# Autodesk Inventor assembly: Wrist_B
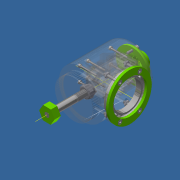
[picture p0: Inventor's stored thumbnail of the model, 180x180]
Saved by Autodesk Inventor 2016 (Build 200138000, 138)
## iProperties
Created: 2015-09-09
Part Number: Wrist_B
Material: Generisch
Document SubType Name: Assembly
Designer: 4ndreas
Mass: 237.443 g
Surface Area: 675.812 cm^2
Volume: 163.226 cm^3
Density: 1.45469 g/cm^3
Author: 4ndreas
## Documents named in this file (14)
- C:\Users\4ndreas\Documents\Inventor\RobotARM v2\v4\_assemblys\WristRot.iam
- C:\Users\4ndreas\Documents\Inventor\Content Center Files\R2014\de-DE\DIN BEARING(1)\DIN 625 SKF - SKF 61807.ipt
- C:\Users\4ndreas\Documents\Inventor\RobotARM v2\v4\_printed parts\60zGelenk.ipt
- C:\Users\4ndreas\Documents\Inventor\RobotARM v2\v4\_motors\[HerkuleX] DRS-010X.iam
- C:\Users\4ndreas\Documents\Inventor\Content Center Files\R2014\de-DE\DIN 912\DIN 912 - M2 x 0,4 x 20 x 19.ipt
- C:\Users\4ndreas\Documents\Inventor\Content Center Files\R2014\de-DE\DIN 912\DIN 912 - M3 x 0,5 x 10 x 8,75.ipt
- C:\Users\4ndreas\Documents\Inventor\Content Center Files\R2014\de-DE\DIN 985\DIN 985 - M8.ipt
- C:\Users\4ndreas\Documents\Inventor\RobotARM v2\v4\_encoder\EncoderMagnet.ipt
- C:\Users\4ndreas\Documents\Inventor\RobotARM v2\v4\_printed parts\Wrist_Cover_2.ipt
- C:\Users\4ndreas\Documents\Inventor\RobotARM v2\v4\_printed parts\magHexMount.ipt
- C:\Users\4ndreas\Documents\Inventor\Content Center Files\R2014\de-DE\DIN 931-1\DIN 931-1 - M8 x 50.ipt
- C:\Users\4ndreas\Documents\Inventor\Content Center Files\R2014\de-DE\DIN 934\DIN 934 - M3 x 0,5.ipt
- C:\Users\4ndreas\Documents\Inventor\RobotARM v2\v4\_printed parts\WristBearingHolder.ipt
- C:\Users\4ndreas\Documents\Inventor\Content Center Files\R2014\de-DE\DIN 7991(2)\DIN 7991 - M3x20.ipt
## Components (25 placed, 13 different names)
1. 60zGelenk:1 — Passend:1, Passend:2, Passend:3, Fluchtend:1, Fluchtend:2, Fluchtend:3, Passend:8, Passend:9, Passend:10, Passend:11, Passend:12, Passend:13, Passend:14, Passend:15, Passend:16, Passend:17, Passend:18, Passend:19, Fluchtend:4, Passend:29, Passend:30, Passend:33, Passend:34, Passend:36, Winkel:2, Passend:38, Passend:39, Passend:45, Passend:46, Passend:48, Passend:49, Passend:50, Passend:51, Passend:52, Passend:53, Passend:54, Passend:55, Passend:56, Fluchtend:8
2. DIN 625 SKF SKF 61807:1 — Passend:1, Passend:2, Passend:4, Passend:29, Passend:30, Passend:62
3. [HerkuleX] DRS-010X:1 [sub-assembly] — Passend:5, Fluchtend:1, Winkel:1
4. DIN 912 - ersetzt durch DIN EN ISO 4762 M2 x 20:1 — Passend:8, Passend:19
5. DIN 912 - ersetzt durch DIN EN ISO 4762 M2 x 20:2 — Passend:9, Passend:18
6. DIN 912 - ersetzt durch DIN EN ISO 4762 M2 x 20:3 — Passend:10, Passend:17
7. DIN 912 - ersetzt durch DIN EN ISO 4762 M2 x 20:4 — Passend:11, Passend:14
8. DIN 912 - ersetzt durch DIN EN ISO 4762 M2 x 20:5 — Passend:13, Passend:16
9. DIN 912 - ersetzt durch DIN EN ISO 4762 M2 x 20:6 — Passend:12, Passend:15
10. DIN 985 - ersetzt durch DIN EN ISO 10511 M8:1 — Passend:38, Passend:39
11. Wrist_Cover_2:1 — Fluchtend:4, Passend:25, Passend:26, Passend:27, Passend:28
12. DIN 912 - ersetzt durch DIN EN ISO 4762 M3 x 10:1 — Passend:26, Passend:27, Passend:33
13. DIN 912 - ersetzt durch DIN EN ISO 4762 M3 x 10:2 — Passend:25, Passend:28, Passend:34
14. EncoderMagnet:1 — Passend:40, Passend:47
15. magHexMount:1 — Passend:42, Passend:43, Passend:44, Passend:47
16. DIN 931-1 - ersetzt durch DIN EN 24014 M8 x 50:1 — Passend:42, Passend:43, Passend:44, Passend:45, Passend:46
17. DIN 934 - ersetzt durch DIN EN 24032/28673/28674 M3:1 — Passend:49, Passend:53, Fluchtend:5
18. DIN 934 - ersetzt durch DIN EN 24032/28673/28674 M3:2 — Passend:50, Passend:54, Fluchtend:6
19. DIN 934 - ersetzt durch DIN EN 24032/28673/28674 M3:3 — Passend:48, Passend:52, Fluchtend:5, Fluchtend:6, Fluchtend:7
20. DIN 934 - ersetzt durch DIN EN 24032/28673/28674 M3:4 — Passend:51, Passend:55, Fluchtend:7, Passend:56
21. WristBearingHolder:1 — Fluchtend:8
22. DIN 7991 M3x20:1
23. DIN 7991 M3x20:2
24. DIN 7991 M3x20:4
25. DIN 7991 M3x20:3
## Relationships (65: Mate 51, Flush 12, Angle 2)
- Passend:1 [Mate]: 60zGelenk:1 ↔ DIN 625 SKF SKF 61807:1
- Passend:2 [Mate]: 60zGelenk:1 ↔ DIN 625 SKF SKF 61807:1
- Passend:3 [Mate]: 60zGelenk:1
- Passend:4 [Mate]: DIN 625 SKF SKF 61807:1
- Passend:5 [Mate]: [HerkuleX] DRS-010X:1
- Fluchtend:1 [Flush] (5 mm): 60zGelenk:1 ↔ [HerkuleX] DRS-010X:1
- Fluchtend:2 [Flush]: 60zGelenk:1
- Winkel:1 [Angle] (90 deg): [HerkuleX] DRS-010X:1
- Fluchtend:3 [Flush]: 60zGelenk:1
- Passend:8 [Mate]: 60zGelenk:1 ↔ DIN 912 - ersetzt durch DIN EN ISO 4762 M2 x 20:1
- Passend:9 [Mate]: 60zGelenk:1 ↔ DIN 912 - ersetzt durch DIN EN ISO 4762 M2 x 20:2
- Passend:10 [Mate]: 60zGelenk:1 ↔ DIN 912 - ersetzt durch DIN EN ISO 4762 M2 x 20:3
- Passend:11 [Mate]: 60zGelenk:1 ↔ DIN 912 - ersetzt durch DIN EN ISO 4762 M2 x 20:4
- Passend:12 [Mate]: 60zGelenk:1 ↔ DIN 912 - ersetzt durch DIN EN ISO 4762 M2 x 20:6
- Passend:13 [Mate]: 60zGelenk:1 ↔ DIN 912 - ersetzt durch DIN EN ISO 4762 M2 x 20:5
- Passend:14 [Mate]: 60zGelenk:1 ↔ DIN 912 - ersetzt durch DIN EN ISO 4762 M2 x 20:4
- Passend:15 [Mate]: 60zGelenk:1 ↔ DIN 912 - ersetzt durch DIN EN ISO 4762 M2 x 20:6
- Passend:16 [Mate]: 60zGelenk:1 ↔ DIN 912 - ersetzt durch DIN EN ISO 4762 M2 x 20:5
- Passend:17 [Mate]: 60zGelenk:1 ↔ DIN 912 - ersetzt durch DIN EN ISO 4762 M2 x 20:3
- Passend:18 [Mate]: 60zGelenk:1 ↔ DIN 912 - ersetzt durch DIN EN ISO 4762 M2 x 20:2
- Passend:19 [Mate]: 60zGelenk:1 ↔ DIN 912 - ersetzt durch DIN EN ISO 4762 M2 x 20:1
- Fluchtend:4 [Flush]: 60zGelenk:1 ↔ Wrist_Cover_2:1
- Passend:25 [Mate]: Wrist_Cover_2:1 ↔ DIN 912 - ersetzt durch DIN EN ISO 4762 M3 x 10:2
- Passend:26 [Mate]: Wrist_Cover_2:1 ↔ DIN 912 - ersetzt durch DIN EN ISO 4762 M3 x 10:1
- Passend:27 [Mate]: Wrist_Cover_2:1 ↔ DIN 912 - ersetzt durch DIN EN ISO 4762 M3 x 10:1
- Passend:28 [Mate]: Wrist_Cover_2:1 ↔ DIN 912 - ersetzt durch DIN EN ISO 4762 M3 x 10:2
- Passend:29 [Mate]: 60zGelenk:1 ↔ DIN 625 SKF SKF 61807:1
- Passend:30 [Mate]: 60zGelenk:1 ↔ DIN 625 SKF SKF 61807:1
- Passend:33 [Mate]: 60zGelenk:1 ↔ DIN 912 - ersetzt durch DIN EN ISO 4762 M3 x 10:1
- Passend:34 [Mate]: 60zGelenk:1 ↔ DIN 912 - ersetzt durch DIN EN ISO 4762 M3 x 10:2
- Passend:35 [Mate]
- Passend:36 [Mate]: 60zGelenk:1
- Winkel:2 [Angle] (0 deg): 60zGelenk:1
- Passend:38 [Mate]: 60zGelenk:1 ↔ DIN 985 - ersetzt durch DIN EN ISO 10511 M8:1
- Passend:39 [Mate]: 60zGelenk:1 ↔ DIN 985 - ersetzt durch DIN EN ISO 10511 M8:1
- Passend:40 [Mate]: EncoderMagnet:1
- Passend:42 [Mate]: magHexMount:1 ↔ DIN 931-1 - ersetzt durch DIN EN 24014 M8 x 50:1
- Passend:43 [Mate]: magHexMount:1 ↔ DIN 931-1 - ersetzt durch DIN EN 24014 M8 x 50:1
- Passend:44 [Mate]: magHexMount:1 ↔ DIN 931-1 - ersetzt durch DIN EN 24014 M8 x 50:1
- Passend:45 [Mate] (26 mm): 60zGelenk:1 ↔ DIN 931-1 - ersetzt durch DIN EN 24014 M8 x 50:1
- Passend:46 [Mate]: 60zGelenk:1 ↔ DIN 931-1 - ersetzt durch DIN EN 24014 M8 x 50:1
- Passend:47 [Mate]: EncoderMagnet:1 ↔ magHexMount:1
- Passend:48 [Mate]: 60zGelenk:1 ↔ DIN 934 - ersetzt durch DIN EN 24032/28673/28674 M3:3
- Passend:49 [Mate]: 60zGelenk:1 ↔ DIN 934 - ersetzt durch DIN EN 24032/28673/28674 M3:1
- Passend:50 [Mate]: 60zGelenk:1 ↔ DIN 934 - ersetzt durch DIN EN 24032/28673/28674 M3:2
- Passend:51 [Mate]: 60zGelenk:1 ↔ DIN 934 - ersetzt durch DIN EN 24032/28673/28674 M3:4
- Passend:52 [Mate]: 60zGelenk:1 ↔ DIN 934 - ersetzt durch DIN EN 24032/28673/28674 M3:3
- Passend:53 [Mate]: 60zGelenk:1 ↔ DIN 934 - ersetzt durch DIN EN 24032/28673/28674 M3:1
- Passend:54 [Mate]: 60zGelenk:1 ↔ DIN 934 - ersetzt durch DIN EN 24032/28673/28674 M3:2
- Passend:55 [Mate]: 60zGelenk:1 ↔ DIN 934 - ersetzt durch DIN EN 24032/28673/28674 M3:4
- Fluchtend:5 [Flush]: DIN 934 - ersetzt durch DIN EN 24032/28673/28674 M3:1 ↔ DIN 934 - ersetzt durch DIN EN 24032/28673/28674 M3:3
- Fluchtend:6 [Flush]: DIN 934 - ersetzt durch DIN EN 24032/28673/28674 M3:2 ↔ DIN 934 - ersetzt durch DIN EN 24032/28673/28674 M3:3
- Fluchtend:7 [Flush]: DIN 934 - ersetzt durch DIN EN 24032/28673/28674 M3:3 ↔ DIN 934 - ersetzt durch DIN EN 24032/28673/28674 M3:4
- Passend:56 [Mate]: 60zGelenk:1 ↔ DIN 934 - ersetzt durch DIN EN 24032/28673/28674 M3:4
- Fluchtend:8 [Flush]: 60zGelenk:1 ↔ WristBearingHolder:1
- [Mate]: WristBearingHolder:1 ↔ DIN 7991 M3x20:1
- [Mate]: WristBearingHolder:1 ↔ DIN 7991 M3x20:4
- [Mate]: WristBearingHolder:1 ↔ DIN 7991 M3x20:2
- [Mate]: WristBearingHolder:1 ↔ DIN 7991 M3x20:3
- [Flush]: WristBearingHolder:1 ↔ DIN 7991 M3x20:1
- [Flush]: WristBearingHolder:1 ↔ DIN 7991 M3x20:2
- [Flush]: WristBearingHolder:1 ↔ DIN 7991 M3x20:3
- [Flush]: WristBearingHolder:1 ↔ DIN 7991 M3x20:4
- [Mate]: DIN 934 - ersetzt durch DIN EN 24032/28673/28674 M3:4 ↔ DIN 7991 M3x20:1
- Passend:62 [Mate]: DIN 625 SKF SKF 61807:1
